# Autodesk Inventor assembly: SpringBlock
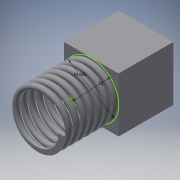
[picture p0: Inventor's stored thumbnail of the model, 180x180]
Saved by Autodesk Inventor 2016 (Build 200138000, 138)
## iProperties
Created: 2015-09-12
Part Number: SpringBlock
Document SubType Name: Assembly
Designer: nightstalker
Author: nightstalker
## Documents named in this file (3)
- C:\Users\nightstalker\Downloads\ENPM 808M\Spring\SpringBlock.iam
- C:\Users\nightstalker\Downloads\ENPM 808M\Spring\Mass.ipt
- C:\Users\nightstalker\Downloads\ENPM 808M\Spring\Spring.ipt
## Components (2 placed, 2 different names)
1. Mass:1 — Rigid:1
2. Spring:1 — Rigid:1
## Relationships (1: WeldJoint 1)
- Rigid:1 [WeldJoint]: Mass:1 ↔ Spring:1
